# Autodesk Inventor assembly: Tensioner
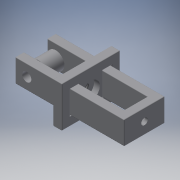
[picture p0: Inventor's stored thumbnail of the model, 180x180]
Saved by Autodesk Inventor 2017 (Build 210142000, 142)
## iProperties
Created: 2017-07-29
Part Number: Tensioner
Document SubType Name: Assembly
Designer: User
Author: User
## Documents named in this file (4)
- C:\Robotics\CAD\2018-19_CAD\Offseason\Tensioner2.iam
- C:\Robotics\CAD\2018-19_CAD\Offseason\TensionerAxleHolder2.ipt
- C:\Robotics\CAD\2018-19_CAD\Offseason\TensionerPlate2.ipt
- C:\Robotics\CAD\2016-17_CAD\Custom COTS\Spacer.188ID.375W.ipt
## Components (3 placed, 3 different names)
1. TensionerAxleHolder2:1 — Mate:1, Flush:1, Flush:2, Insert:1
2. TensionerPlate2:1 — Mate:1, Flush:1, Flush:2
3. Spacer.188ID.375W:1 — Insert:1
## Relationships (4: Flush 2, Mate 1, Insert 1)
- Mate:1: TensionerAxleHolder2:1 ↔ TensionerPlate2:1
- Flush:1 (4.7625 mm): TensionerAxleHolder2:1 ↔ TensionerPlate2:1
- Flush:2 (-29.21 mm): TensionerAxleHolder2:1 ↔ TensionerPlate2:1
- Insert:1 (1.5875 mm): TensionerAxleHolder2:1 ↔ Spacer.188ID.375W:1
